# Autodesk Inventor assembly: SP
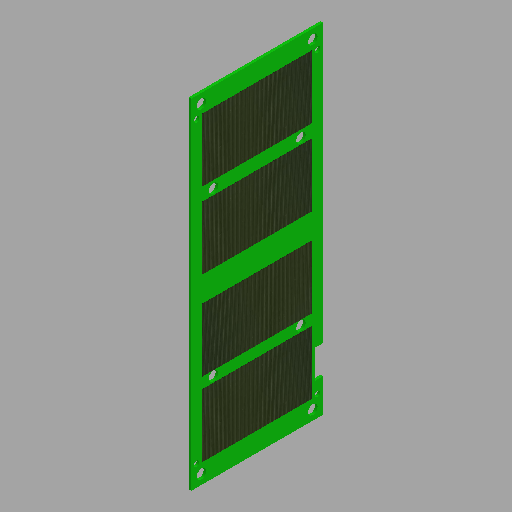
[picture p0: Inventor's stored thumbnail of the model, 512x512]
Saved by Autodesk Inventor 2022 (Build 260153000, 153)
## iProperties
Created: 2021-09-09
Part Number: SP
Document SubType Name: Assembly
Designer: Bowen O'Steen
Author: Bowen O'Steen
## Documents named in this file (3)
- C:\Users\gwhen\OneDrive\Desktop\Vault\Designs\MEMESat\MemeSat\Engineering Data\MemeSat\Solar Panels\SP.iam
- C:\Users\gwhen\OneDrive\Desktop\Vault\Designs\MEMESat\MemeSat\Engineering Data\MemeSat\Solar Panels\SolarPCB.ipt
- C:\Users\gwhen\OneDrive\Desktop\Vault\Designs\MEMESat\MemeSat\Engineering Data\MemeSat\Solar Panels\QJcell.ipt
## Components (5 placed, 2 different names)
1. SolarPCB:1 — Mate:1, Mate:2, Flush:1, Mate:3, Mate:4, Angle:1, Angle:2, Mate:5, Flush:2, Mate:7, Mate:8, Flush:4, Mate:9, Mate:10, Flush:5, Mate:12
2. QJcell:1 — Mate:3, Angle:1, Flush:2, Mate:12
3. QJcell:2 — Mate:4, Angle:2, Mate:5, Mate:11
4. QJcell:3 — Mate:7, Mate:8, Flush:4, Mate:11
5. QJcell:4 — Mate:9, Mate:10, Flush:5
## Relationships (17: Mate 11, Flush 4, Angle 2)
- Mate:1: SolarPCB:1
- Mate:2: SolarPCB:1
- Flush:1: SolarPCB:1
- Mate:3: SolarPCB:1 ↔ QJcell:1
- Mate:4: SolarPCB:1 ↔ QJcell:2
- Angle:1 (0 deg): SolarPCB:1 ↔ QJcell:1
- Angle:2 (0 deg): SolarPCB:1 ↔ QJcell:2
- Mate:5: SolarPCB:1 ↔ QJcell:2
- Flush:2: SolarPCB:1 ↔ QJcell:1
- Mate:7: SolarPCB:1 ↔ QJcell:3
- Mate:8: SolarPCB:1 ↔ QJcell:3
- Flush:4 (11.5 mm): SolarPCB:1 ↔ QJcell:3
- Mate:9: SolarPCB:1 ↔ QJcell:4
- Mate:10: SolarPCB:1 ↔ QJcell:4
- Flush:5 (12.25 mm): SolarPCB:1 ↔ QJcell:4
- Mate:11 (8.25 mm): QJcell:2 ↔ QJcell:3
- Mate:12 (115 mm): SolarPCB:1 ↔ QJcell:1
